# Autodesk Inventor assembly: WheelSuspension
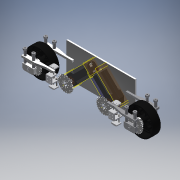
[picture p0: Inventor's stored thumbnail of the model, 180x180]
Saved by Autodesk Inventor 2017 (Build 210142000, 142)
## iProperties
Created: 2018-05-04
Part Number: WheelSuspension
Document SubType Name: Assembly
Designer: User
Author: User
## Documents named in this file (26)
- C:\Robotics\CAD\2018-19_CAD\Offseason\WheelSuspension.iam
- C:\Robotics\CAD\COTSParts\Wheels\4in Wheel Intergreated Hub 8mm Rev2.ipt
- C:\Robotics\CAD\2016-17_CAD\Custom COTS\4inax.ipt
- C:\Robotics\CAD\2018-19_CAD\Offseason\WheelSuspensionHub.ipt
- C:\Robotics\CAD\COTSParts\Actobotics\535 parts\535198Bearing.25ID.5OD.ipt
- C:\Robotics\CAD\2018-19_CAD\Offseason\WheelandSprocketComboHub2.ipt
- C:\Robotics\CAD\COTSParts\Actobotics\615 parts\615106Sprocket.5inBore.25inPitch24Teeth.ipt
- C:\Robotics\CAD\2018-19_CAD\Offseason\WheelSuspensionFork.ipt
- C:\Robotics\CAD\2018-19_CAD\Offseason\SuspensionDrivePlate.ipt
- C:\Robotics\CAD\COTSParts\Rev\REV-41-1300HexMotor.ipt
- C:\Robotics\CAD\COTSParts\Rev\REV-41-1349HexAxle.ipt
- C:\Robotics\CAD\COTSParts\Fasteners\91259A587_ALLOY STEEL SHOULDER SCREW.ipt
- C:\Robotics\CAD\2018-19_CAD\Offseason\Tensioner4b.iam
- C:\Robotics\CAD\2018-19_CAD\Offseason\Tensioner4a.iam
- C:\Robotics\CAD\COTSParts\Wheels\4in Wheel Intergreated Hub 8mm Rev21_MIR.ipt
- C:\Robotics\CAD\2016-17_CAD\Custom COTS\4inax1_MIR.ipt
- C:\Robotics\CAD\2018-19_CAD\Offseason\WheelSuspensionHub1_MIR.ipt
- C:\Robotics\CAD\COTSParts\Actobotics\535 parts\535198Bearing.25ID.5OD1_MIR.ipt
- C:\Robotics\CAD\2018-19_CAD\Offseason\WheelandSprocketComboHub21_MIR.ipt
- C:\Robotics\CAD\COTSParts\Actobotics\615 parts\615106Sprocket.5inBore.25inPitch24Teeth1_MIR.ipt
- C:\Robotics\CAD\2018-19_CAD\Offseason\WheelSuspensionFork1_MIR.ipt
- C:\Robotics\CAD\COTSParts\Rev\REV-41-1300HexMotor1_MIR.ipt
- C:\Robotics\CAD\COTSParts\Rev\REV-41-1349HexAxle1_MIR.ipt
- C:\Robotics\CAD\COTSParts\Fasteners\91259A587_ALLOY STEEL SHOULDER SCREW1_MIR.ipt
- C:\Robotics\CAD\2018-19_CAD\Offseason\Tensioner4b1_MIR.iam
- C:\Robotics\CAD\2018-19_CAD\Offseason\Tensioner4a1_MIR.iam
## Components (41 placed, 25 different names)
1. 4in Wheel Intergreated Hub 8mm Rev2:1 — Insert:6, Insert:46
2. 4inax:1 — Insert:2
3. WheelSuspensionHub:1 — Insert:1, Mate:2, Insert:10, Insert:38, Insert:39
4. 535198Bearing.25ID.5OD:1 — Insert:1, Insert:2
5. WheelandSprocketComboHub2:1 — Insert:5, Insert:6, Insert:10
6. 615106Sprocket.5inBore.25inPitch24Teeth:1 — Insert:5, Flush:29
7. WheelSuspensionHub:2 — Insert:7, Insert:37, Insert:40, Insert:46
8. 535198Bearing.25ID.5OD:2 — Insert:7, Mate:2
9. WheelSuspensionFork:1 — Insert:41, Insert:42, Mate:54, Mate:55
10. SuspensionDrivePlate:1 — Mate:50, Mate:51, Flush:32, Insert:43, Insert:44, Flush:34, Mate:58
11. SuspensionDrivePlate:2 — Mate:6, Flush:1, Flush:2, Mate:27, Mate:28, Flush:24, Angle:8, Mate:36, Mate:37, Mate:38, Insert:41, Insert:42, Flush:32
12. REV-41-1300HexMotor:1 — Mate:27, Mate:28, Flush:24
13. REV-41-1300HexMotor:2 — Angle:8, Mate:36, Mate:37, Mate:38, Mate:39, Mate:40, Flush:28
14. 615106Sprocket.5inBore.25inPitch24Teeth:5 — Mate:41, Flush:29
15. REV-41-1349HexAxle:3 — Mate:39, Mate:40, Flush:28, Mate:41
16. 91259A587_ALLOY STEEL SHOULDER SCREW:1 — Insert:39, Mate:56
17. 91259A587_ALLOY STEEL SHOULDER SCREW:2 — Insert:37, Mate:54
18. 91259A587_ALLOY STEEL SHOULDER SCREW:3 — Insert:40, Mate:55
19. 91259A587_ALLOY STEEL SHOULDER SCREW:4 — Insert:38, Insert:45
20. Tensioner4b:1 [sub-assembly] — Mate:51, Mate:57, Flush:33, Mate:58
21. Tensioner4a:1 [sub-assembly] — Mate:50, Mate:57, Flush:33, Flush:34
22. WheelSuspensionFork:2 — Insert:43, Insert:44, Mate:56, Insert:45
23. 4in Wheel Intergreated Hub 8mm Rev21_MIR:1 — Insert:50, Insert:52
24. 4inax1_MIR:1 — Insert:47
25. WheelSuspensionHub1_MIR:1 — Insert:48, Insert:49, Mate:59, Insert:54, Insert:57
26. 535198Bearing.25ID.5OD1_MIR:1 — Insert:47, Insert:48
27. WheelandSprocketComboHub21_MIR:1 — Insert:49, Insert:50, Insert:51
28. 615106Sprocket.5inBore.25inPitch24Teeth1_MIR:1 — Insert:51, Flush:35
29. WheelSuspensionHub1_MIR:2 — Insert:52, Insert:53, Insert:55, Insert:56
30. 535198Bearing.25ID.5OD1_MIR:2 — Mate:59, Insert:53
31. WheelSuspensionFork1_MIR:1 — Mate:63, Mate:64
32. REV-41-1300HexMotor1_MIR:1 — Flush:36, Mate:61, Mate:62
33. 615106Sprocket.5inBore.25inPitch24Teeth1_MIR:2 — Flush:35, Mate:60
34. REV-41-1349HexAxle1_MIR:1 — Mate:60, Flush:36, Mate:61, Mate:62
35. 91259A587_ALLOY STEEL SHOULDER SCREW1_MIR:1 — Insert:54, Mate:66
36. 91259A587_ALLOY STEEL SHOULDER SCREW1_MIR:2 — Mate:63, Insert:55
37. 91259A587_ALLOY STEEL SHOULDER SCREW1_MIR:3 — Mate:64, Insert:56
38. 91259A587_ALLOY STEEL SHOULDER SCREW1_MIR:4 — Insert:57, Insert:58
39. Tensioner4b1_MIR:1 [sub-assembly] — Flush:37, Mate:65
40. Tensioner4a1_MIR:1 [sub-assembly] — Flush:37, Mate:65
41. WheelSuspensionFork1_MIR:2 — Insert:58, Mate:66
## Relationships (65: Insert 28, Mate 25, Flush 11, Angle 1)
- Insert:1: WheelSuspensionHub:1 ↔ 535198Bearing.25ID.5OD:1
- Insert:2 (3.175 mm): 4inax:1 ↔ 535198Bearing.25ID.5OD:1
- Insert:5: WheelandSprocketComboHub2:1 ↔ 615106Sprocket.5inBore.25inPitch24Teeth:1
- Insert:6: 4in Wheel Intergreated Hub 8mm Rev2:1 ↔ WheelandSprocketComboHub2:1
- Insert:7: WheelSuspensionHub:2 ↔ 535198Bearing.25ID.5OD:2
- Mate:2: WheelSuspensionHub:1 ↔ 535198Bearing.25ID.5OD:2
- Insert:10 (3.175 mm): WheelSuspensionHub:1 ↔ WheelandSprocketComboHub2:1
- Mate:6: SuspensionDrivePlate:2
- Flush:1: SuspensionDrivePlate:2
- Flush:2: SuspensionDrivePlate:2
- Mate:27: SuspensionDrivePlate:2 ↔ REV-41-1300HexMotor:1
- Mate:28 (-3.175 mm): SuspensionDrivePlate:2 ↔ REV-41-1300HexMotor:1
- Flush:24 (12.7 mm): SuspensionDrivePlate:2 ↔ REV-41-1300HexMotor:1
- Angle:8 (135 deg): SuspensionDrivePlate:2 ↔ REV-41-1300HexMotor:2
- Mate:36 (-34.925 mm): SuspensionDrivePlate:2 ↔ REV-41-1300HexMotor:2
- Mate:37: SuspensionDrivePlate:2 ↔ REV-41-1300HexMotor:2
- Mate:38 (-50.8 mm): SuspensionDrivePlate:2 ↔ REV-41-1300HexMotor:2
- Mate:39: REV-41-1300HexMotor:2 ↔ REV-41-1349HexAxle:3
- Mate:40: REV-41-1300HexMotor:2 ↔ REV-41-1349HexAxle:3
- Flush:28 (-25.4 mm): REV-41-1300HexMotor:2 ↔ REV-41-1349HexAxle:3
- Mate:41: 615106Sprocket.5inBore.25inPitch24Teeth:5 ↔ REV-41-1349HexAxle:3
- Flush:29: 615106Sprocket.5inBore.25inPitch24Teeth:1 ↔ 615106Sprocket.5inBore.25inPitch24Teeth:5
- Insert:37: WheelSuspensionHub:2 ↔ 91259A587_ALLOY STEEL SHOULDER SCREW:2
- Insert:38: WheelSuspensionHub:1 ↔ 91259A587_ALLOY STEEL SHOULDER SCREW:4
- Insert:39: WheelSuspensionHub:1 ↔ 91259A587_ALLOY STEEL SHOULDER SCREW:1
- Insert:40: WheelSuspensionHub:2 ↔ 91259A587_ALLOY STEEL SHOULDER SCREW:3
- Mate:50: SuspensionDrivePlate:1 ↔ Tensioner4a:1
- Mate:51: SuspensionDrivePlate:1 ↔ Tensioner4b:1
- Insert:41: WheelSuspensionFork:1 ↔ SuspensionDrivePlate:2
- Insert:42: WheelSuspensionFork:1 ↔ SuspensionDrivePlate:2
- Mate:54: WheelSuspensionFork:1 ↔ 91259A587_ALLOY STEEL SHOULDER SCREW:2
- Mate:55: WheelSuspensionFork:1 ↔ 91259A587_ALLOY STEEL SHOULDER SCREW:3
- Flush:32: SuspensionDrivePlate:1 ↔ SuspensionDrivePlate:2
- Insert:43: SuspensionDrivePlate:1 ↔ WheelSuspensionFork:2
- Insert:44: SuspensionDrivePlate:1 ↔ WheelSuspensionFork:2
- Mate:56: 91259A587_ALLOY STEEL SHOULDER SCREW:1 ↔ WheelSuspensionFork:2
- Insert:45 (15.875 mm): 91259A587_ALLOY STEEL SHOULDER SCREW:4 ↔ WheelSuspensionFork:2
- Insert:46 (9.525 mm): 4in Wheel Intergreated Hub 8mm Rev2:1 ↔ WheelSuspensionHub:2
- Mate:57: Tensioner4b:1 ↔ Tensioner4a:1
- Flush:33: Tensioner4b:1 ↔ Tensioner4a:1
- Flush:34: SuspensionDrivePlate:1 ↔ Tensioner4a:1
- Mate:58 (-34.925 mm): SuspensionDrivePlate:1 ↔ Tensioner4b:1
- Insert:47 (3.175 mm): 4inax1_MIR:1 ↔ 535198Bearing.25ID.5OD1_MIR:1
- Insert:48: WheelSuspensionHub1_MIR:1 ↔ 535198Bearing.25ID.5OD1_MIR:1
- Insert:49 (3.175 mm): WheelSuspensionHub1_MIR:1 ↔ WheelandSprocketComboHub21_MIR:1
- Insert:50: 4in Wheel Intergreated Hub 8mm Rev21_MIR:1 ↔ WheelandSprocketComboHub21_MIR:1
- Insert:51: WheelandSprocketComboHub21_MIR:1 ↔ 615106Sprocket.5inBore.25inPitch24Teeth1_MIR:1
- Insert:52 (9.525 mm): 4in Wheel Intergreated Hub 8mm Rev21_MIR:1 ↔ WheelSuspensionHub1_MIR:2
- Mate:59: WheelSuspensionHub1_MIR:1 ↔ 535198Bearing.25ID.5OD1_MIR:2
- Insert:53: WheelSuspensionHub1_MIR:2 ↔ 535198Bearing.25ID.5OD1_MIR:2
- Flush:35: 615106Sprocket.5inBore.25inPitch24Teeth1_MIR:1 ↔ 615106Sprocket.5inBore.25inPitch24Teeth1_MIR:2
- Mate:60: 615106Sprocket.5inBore.25inPitch24Teeth1_MIR:2 ↔ REV-41-1349HexAxle1_MIR:1
- Flush:36 (-25.4 mm): REV-41-1300HexMotor1_MIR:1 ↔ REV-41-1349HexAxle1_MIR:1
- Mate:61: REV-41-1300HexMotor1_MIR:1 ↔ REV-41-1349HexAxle1_MIR:1
- Mate:62: REV-41-1300HexMotor1_MIR:1 ↔ REV-41-1349HexAxle1_MIR:1
- Insert:54: WheelSuspensionHub1_MIR:1 ↔ 91259A587_ALLOY STEEL SHOULDER SCREW1_MIR:1
- Mate:63: WheelSuspensionFork1_MIR:1 ↔ 91259A587_ALLOY STEEL SHOULDER SCREW1_MIR:2
- Insert:55: WheelSuspensionHub1_MIR:2 ↔ 91259A587_ALLOY STEEL SHOULDER SCREW1_MIR:2
- Mate:64: WheelSuspensionFork1_MIR:1 ↔ 91259A587_ALLOY STEEL SHOULDER SCREW1_MIR:3
- Insert:56: WheelSuspensionHub1_MIR:2 ↔ 91259A587_ALLOY STEEL SHOULDER SCREW1_MIR:3
- Insert:57: WheelSuspensionHub1_MIR:1 ↔ 91259A587_ALLOY STEEL SHOULDER SCREW1_MIR:4
- Flush:37: Tensioner4b1_MIR:1 ↔ Tensioner4a1_MIR:1
- Mate:65: Tensioner4b1_MIR:1 ↔ Tensioner4a1_MIR:1
- Insert:58 (15.875 mm): 91259A587_ALLOY STEEL SHOULDER SCREW1_MIR:4 ↔ WheelSuspensionFork1_MIR:2
- Mate:66: 91259A587_ALLOY STEEL SHOULDER SCREW1_MIR:1 ↔ WheelSuspensionFork1_MIR:2
